# Autodesk Inventor assembly: SansCapacFata
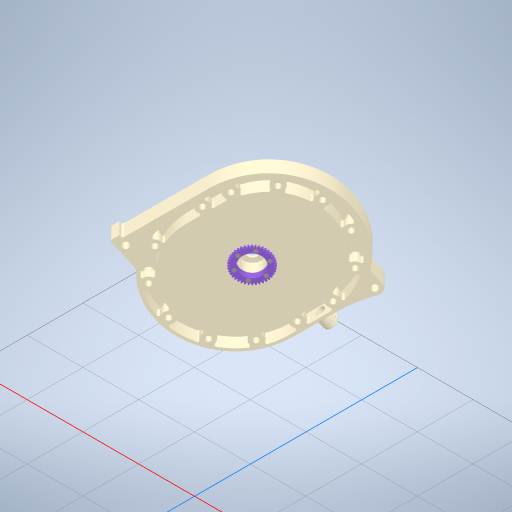
[picture p0: Inventor's stored thumbnail of the model, 512x512]
Saved by Autodesk Inventor 2024 (Build 280153000, 153)
## iProperties
Created: 2024-05-18
Part Number: SansCapacFata
Document SubType Name: Assembly
Designer: alexa
Author: alexa
## Documents named in this file (4)
- C:\Users\alexa\OneDrive\Documents\ANUL I\SEM 2\CAD\Tituleasa Ioana\SansCapacFata.iam
- C:\Users\alexa\OneDrive\Documents\ANUL I\SEM 2\CAD\Fisiere auxiliare teme Inventor\Fisiere auxiliare teme Inventor\7 - Wankel\CapacFata.ipt
- C:\Users\alexa\OneDrive\Documents\ANUL I\SEM 2\CAD\Fisiere auxiliare teme Inventor\Fisiere auxiliare teme Inventor\7 - Wankel\Pinion.ipt
- C:\Users\alexa\OneDrive\Documents\ANUL I\SEM 2\CAD\Tituleasa Ioana\Subans-M4x10.iam
## Components (3 placed, 3 different names)
1. CapacFata:1 — Mate:1, Mate:2, Angle:1
2. Pinion:1 — Mate:1, Mate:2, Angle:1
3. Subans-M4x10:1 [sub-assembly]
## Relationships (4: Mate 2, Angle 1, Insert 1)
- Mate:1: CapacFata:1 ↔ Pinion:1
- Mate:2: CapacFata:1 ↔ Pinion:1
- Angle:1 (99 deg): CapacFata:1 ↔ Pinion:1
- [Insert]: Pinion:1 ↔ Subans-M4x10:1
